# Autodesk Inventor assembly: Competition VEX unit
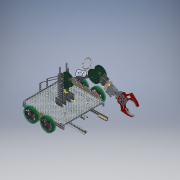
[picture p0: Inventor's stored thumbnail of the model, 180x180]
Saved by Autodesk Inventor 2018 (Build 220112000, 112)
## iProperties
Created: 2018-11-09
Part Number: Competition VEX unit
Document SubType Name: Assembly
Designer: USER
Author: USER
## Documents named in this file (18)
- C:\Users\USER\Desktop\School\Grade 12\Sem 1\Computer Engineering\Competition Robot Inventor\Competition VEX unit.iam
- C:\Users\USER\Downloads\Inventor_2013_VEX_ KOP_-_Metric\Metric\Structure\Chassis Rail 25 Hole.ipt
- C:\Users\USER\Downloads\Inventor_2013_VEX_ KOP_-_Metric\Metric\Structure\Chassis Rail 16 Hole.ipt
- C:\Users\USER\Downloads\Inventor_2013_VEX_ KOP_-_Metric\Metric\Structure\Plate 5x25 Hole.ipt
- C:\Users\USER\Downloads\Inventor_2013_VEX_ KOP_-_Metric\Metric\Structure\Bar 1x25.ipt
- C:\Users\USER\Downloads\Inventor_2013_VEX_ KOP_-_Metric\Metric\Motion\Bearing Flat.ipt
- C:\Users\USER\Downloads\Inventor_2013_VEX_ KOP_-_Metric\Metric\Motion\60 Tooth Gear.ipt
- C:\Users\USER\Downloads\Inventor_2013_VEX_ KOP_-_Metric\Metric\Motion\Shaft 4 inch.ipt
- C:\Users\USER\Downloads\Inventor_2013_VEX_ KOP_-_Metric\Metric\Motion\4 inch Wheel.iam
- C:\Users\USER\Downloads\Inventor_2013_VEX_ KOP_-_Metric\Metric\Structure\C-Channel 1x2x1x15 Hole.ipt
- C:\Users\USER\Downloads\Inventor_2013_VEX_ KOP_-_Metric\Metric\Structure\C-Channel 1x2x1x25 Hole.ipt
- C:\Users\USER\Downloads\Inventor_2013_VEX_ KOP_-_Metric\Metric\Motion\19 Tooth Rack Gear.ipt
- C:\Users\USER\Downloads\Inventor_2013_VEX_ KOP_-_Metric\Metric\Motion\Shaft 3 inch.ipt
- C:\Users\USER\Downloads\Inventor_2013_VEX_ KOP_-_Metric\Metric\Motion\Shaft Collar.iam
- C:\Users\USER\Downloads\Inventor_2013_VEX_ KOP_-_Metric\Metric\Structure\Lin Mot-Rack Brk.ipt
- C:\Users\USER\Downloads\Inventor_2013_VEX_ KOP_-_Metric\Metric\Structure\Chassis Bumper 15 Hole.ipt
- C:\Users\USER\Downloads\Inventor_2013_VEX_ KOP_-_Metric\Metric\Motion\12 Tooth Gear.ipt
- C:\Users\USER\Downloads\Inventor_2013_VEX_ KOP_-_Metric\Metric\Structure\Bar 1x20.ipt
## Components (58 placed, 18 different names)
1. Chassis Rail 25 Hole:1 — Rigid:3, Rigid:27
2. Chassis Rail 25 Hole:2 — Rigid:1, Rigid:2, Rigid:28
3. Chassis Rail 25 Hole:3 — Rigid:2, Rigid:4, Rigid:5, Rigid:6, Rigid:7, Rigid:48
4. Chassis Rail 25 Hole:4 — Rigid:1, Rigid:3
5. Plate 5x25 Hole:1 — Rigid:4, Rigid:9, Rigid:38, Rigid:39
6. Plate 5x25 Hole:2 — Rigid:5, Rigid:40
7. Plate 5x25 Hole:3 — Rigid:6, Rigid:41
8. Plate 5x25 Hole:4 — Rigid:7, Rigid:10
9. Bar 1x25:1 — Rigid:46
10. Chassis Rail 16 Hole:1 — Rigid:9, Rigid:11, Rigid:12, Rigid:13
11. Chassis Rail 16 Hole:2 — Rigid:10, Rigid:14, Rigid:15, Rigid:16
12. Bearing Flat:1 — Rigid:11, Rotational:4
13. Bearing Flat:2 — Rigid:12, Rotational:5
14. Bearing Flat:3 — Rigid:14, Rotational:1
15. Bearing Flat:4 — Rigid:13, Rotational:6
16. Bearing Flat:5 — Rigid:15, Rotational:2
17. Bearing Flat:6 — Rigid:16, Rotational:3
18. 60 Tooth Gear:1 — Rigid:17, Rotation:1
19. 60 Tooth Gear:2 — Rigid:18, Rotation:1, Rotation:2
20. 60 Tooth Gear:3 — Rigid:19, Rotation:2
21. 60 Tooth Gear:4 — Rigid:25, Rotation:4
22. 60 Tooth Gear:5 — Rigid:24, Rotation:3, Rotation:4
23. 60 Tooth Gear:6 — Rigid:23, Rotation:3
24. Shaft 4 inch:1 — Rotational:1, Rigid:17, Rigid:20
25. Shaft 4 inch:2 — Rotational:2, Rigid:18
26. Shaft 4 inch:3 — Rotational:3, Rigid:19, Rigid:21
27. Shaft 4 inch:4 — Rotational:4, Rigid:23, Rigid:22
28. Shaft 4 inch:5 — Rotational:5, Rigid:24
29. Shaft 4 inch:6 — Rotational:6, Rigid:25, Rigid:26
30. 4 inch Wheel:1 [sub-assembly] — Rigid:20
31. 4 inch Wheel:2 [sub-assembly] — Rigid:22
32. 4 inch Wheel:3 [sub-assembly] — Rigid:26
33. 4 inch Wheel:4 [sub-assembly] — Rigid:21
34. C-Channel 1x2x1x15 Hole:1 — Rigid:27
35. Plate 5x25 Hole:5 — Rigid:28, Rigid:29
36. C-Channel 1x2x1x25 Hole:1 — Rigid:29
37. C-Channel 1x2x1x15 Hole:2 — Rigid:30, Rigid:33
38. C-Channel 1x2x1x15 Hole:3 — Rigid:31, Rigid:32
39. 19 Tooth Rack Gear:1 — Rigid:30
40. 19 Tooth Rack Gear:2 — Rigid:31
41. 60 Tooth Gear:7 — Rigid:35, Rotation:6
42. 60 Tooth Gear:8 — Rigid:37, Rotation:6
43. Bearing Flat:7 — Rigid:32, Rigid:34
44. Bearing Flat:8 — Rigid:33, Rigid:36
45. Shaft 3 inch:1 — Rigid:34, Rigid:35, Rotational:7
46. Shaft 3 inch:2 — Rigid:36, Rigid:37, Rotational:8
47. Shaft Collar:1 [sub-assembly] — Rigid:38, Rotational:7
48. Shaft Collar:2 [sub-assembly] — Rigid:39, Rotational:8
49. Lin Mot-Rack Brk:1 — Rigid:40, Rigid:42
50. Lin Mot-Rack Brk:2 — Rigid:41, Rigid:43
51. Chassis Bumper 15 Hole:1 — Rigid:42, Rotational:9, Rigid:46
52. Chassis Bumper 15 Hole:2 — Rigid:43, Rigid:47, Rotational:10
53. Shaft 4 inch:7 — Rigid:44, Rigid:45, Rotational:9
54. 12 Tooth Gear:1 — Rigid:44, Rotation:5
55. 12 Tooth Gear:2 — Rigid:45
56. Bar 1x25:2 — Rigid:47
57. Bar 1x20:1 — Rigid:48
58. Arm Manipulator:1 [sub-assembly] — Rotation:5, Rotational:10
## Relationships (63: WeldJoint 47, RevoluteJoint 10, RelateRotation 6)
- Rigid:1 [WeldJoint]: Chassis Rail 25 Hole:2 ↔ Chassis Rail 25 Hole:4
- Rigid:2 [WeldJoint]: Chassis Rail 25 Hole:2 ↔ Chassis Rail 25 Hole:3
- Rigid:3 [WeldJoint]: Chassis Rail 25 Hole:1 ↔ Chassis Rail 25 Hole:4
- Rigid:4 [WeldJoint]: Chassis Rail 25 Hole:3 ↔ Plate 5x25 Hole:1
- Rigid:5 [WeldJoint]: Chassis Rail 25 Hole:3 ↔ Plate 5x25 Hole:2
- Rigid:6 [WeldJoint]: Chassis Rail 25 Hole:3 ↔ Plate 5x25 Hole:3
- Rigid:7 [WeldJoint]: Chassis Rail 25 Hole:3 ↔ Plate 5x25 Hole:4
- Rigid:9 [WeldJoint]: Plate 5x25 Hole:1 ↔ Chassis Rail 16 Hole:1
- Rigid:10 [WeldJoint]: Plate 5x25 Hole:4 ↔ Chassis Rail 16 Hole:2
- Rigid:11 [WeldJoint]: Chassis Rail 16 Hole:1 ↔ Bearing Flat:1
- Rigid:12 [WeldJoint]: Chassis Rail 16 Hole:1 ↔ Bearing Flat:2
- Rigid:13 [WeldJoint]: Chassis Rail 16 Hole:1 ↔ Bearing Flat:4
- Rigid:14 [WeldJoint]: Chassis Rail 16 Hole:2 ↔ Bearing Flat:3
- Rigid:15 [WeldJoint]: Chassis Rail 16 Hole:2 ↔ Bearing Flat:5
- Rigid:16 [WeldJoint]: Chassis Rail 16 Hole:2 ↔ Bearing Flat:6
- Rotational:1 [RevoluteJoint] (25.4 mm): Bearing Flat:3 ↔ Shaft 4 inch:1
- Rotational:2 [RevoluteJoint] (25.4 mm): Bearing Flat:5 ↔ Shaft 4 inch:2
- Rotational:3 [RevoluteJoint] (-25.4 mm): Bearing Flat:6 ↔ Shaft 4 inch:3
- Rigid:17 [WeldJoint] (25.4 mm): 60 Tooth Gear:1 ↔ Shaft 4 inch:1
- Rigid:18 [WeldJoint] (-25.4 mm): 60 Tooth Gear:2 ↔ Shaft 4 inch:2
- Rigid:19 [WeldJoint] (-25.4 mm): 60 Tooth Gear:3 ↔ Shaft 4 inch:3
- Rotation:1 [RelateRotation] (1 ul): 60 Tooth Gear:1 ↔ 60 Tooth Gear:2
- Rotation:2 [RelateRotation] (1 ul): 60 Tooth Gear:2 ↔ 60 Tooth Gear:3
- Rigid:20 [WeldJoint] (20.32 mm): Shaft 4 inch:1 ↔ 4 inch Wheel:1
- Rigid:21 [WeldJoint] (20.32 mm): Shaft 4 inch:3 ↔ 4 inch Wheel:4
- Rotational:4 [RevoluteJoint] (-25.4 mm): Bearing Flat:1 ↔ Shaft 4 inch:4
- Rotational:5 [RevoluteJoint] (-25.4 mm): Bearing Flat:2 ↔ Shaft 4 inch:5
- Rotational:6 [RevoluteJoint] (-25.4 mm): Bearing Flat:4 ↔ Shaft 4 inch:6
- Rigid:23 [WeldJoint] (-25.4 mm): 60 Tooth Gear:6 ↔ Shaft 4 inch:4
- Rigid:24 [WeldJoint] (-25.4 mm): 60 Tooth Gear:5 ↔ Shaft 4 inch:5
- Rigid:25 [WeldJoint] (-25.4 mm): 60 Tooth Gear:4 ↔ Shaft 4 inch:6
- Rotation:3 [RelateRotation] (1 ul): 60 Tooth Gear:5 ↔ 60 Tooth Gear:6
- Rotation:4 [RelateRotation] (1 ul): 60 Tooth Gear:4 ↔ 60 Tooth Gear:5
- Rigid:22 [WeldJoint]: Shaft 4 inch:4 ↔ 4 inch Wheel:2
- Rigid:26 [WeldJoint]: Shaft 4 inch:6 ↔ 4 inch Wheel:3
- Rigid:27 [WeldJoint]: Chassis Rail 25 Hole:1 ↔ C-Channel 1x2x1x15 Hole:1
- Rigid:28 [WeldJoint]: Chassis Rail 25 Hole:2 ↔ Plate 5x25 Hole:5
- Rigid:29 [WeldJoint]: Plate 5x25 Hole:5 ↔ C-Channel 1x2x1x25 Hole:1
- Rigid:30 [WeldJoint]: C-Channel 1x2x1x15 Hole:2 ↔ 19 Tooth Rack Gear:1
- Rigid:31 [WeldJoint]: C-Channel 1x2x1x15 Hole:3 ↔ 19 Tooth Rack Gear:2
- Rigid:32 [WeldJoint]: C-Channel 1x2x1x15 Hole:3 ↔ Bearing Flat:7
- Rigid:33 [WeldJoint]: C-Channel 1x2x1x15 Hole:2 ↔ Bearing Flat:8
- Rigid:34 [WeldJoint]: Bearing Flat:7 ↔ Shaft 3 inch:1
- Rigid:35 [WeldJoint] (43.18 mm): 60 Tooth Gear:7 ↔ Shaft 3 inch:1
- Rigid:36 [WeldJoint]: Bearing Flat:8 ↔ Shaft 3 inch:2
- Rigid:37 [WeldJoint] (-43.18 mm): 60 Tooth Gear:8 ↔ Shaft 3 inch:2
- Rigid:38 [WeldJoint]: Plate 5x25 Hole:1 ↔ Shaft Collar:1
- Rigid:39 [WeldJoint]: Plate 5x25 Hole:1 ↔ Shaft Collar:2
- Rotational:7 [RevoluteJoint] (25.4 mm): Shaft 3 inch:1 ↔ Shaft Collar:1
- Rotational:8 [RevoluteJoint] (25.4 mm): Shaft 3 inch:2 ↔ Shaft Collar:2
- Rigid:40 [WeldJoint]: Plate 5x25 Hole:2 ↔ Lin Mot-Rack Brk:1
- Rigid:41 [WeldJoint]: Plate 5x25 Hole:3 ↔ Lin Mot-Rack Brk:2
- Rigid:42 [WeldJoint]: Lin Mot-Rack Brk:1 ↔ Chassis Bumper 15 Hole:1
- Rigid:43 [WeldJoint]: Lin Mot-Rack Brk:2 ↔ Chassis Bumper 15 Hole:2
- Rigid:44 [WeldJoint] (-38.1 mm): Shaft 4 inch:7 ↔ 12 Tooth Gear:1
- Rigid:45 [WeldJoint] (-25.4 mm): Shaft 4 inch:7 ↔ 12 Tooth Gear:2
- Rotational:9 [RevoluteJoint] (-25.4 mm): Chassis Bumper 15 Hole:1 ↔ Shaft 4 inch:7
- Rigid:46 [WeldJoint]: Bar 1x25:1 ↔ Chassis Bumper 15 Hole:1
- Rigid:47 [WeldJoint]: Chassis Bumper 15 Hole:2 ↔ Bar 1x25:2
- Rigid:48 [WeldJoint]: Chassis Rail 25 Hole:3 ↔ Bar 1x20:1
- Rotation:5 [RelateRotation] (1 ul): 12 Tooth Gear:1 ↔ Arm Manipulator:1
- Rotational:10 [RevoluteJoint] (-33.02 mm): Chassis Bumper 15 Hole:2 ↔ Arm Manipulator:1
- Rotation:6 [RelateRotation] (1 ul): 60 Tooth Gear:7 ↔ 60 Tooth Gear:8
